# Autodesk Inventor assembly: Slidey Mecanum L thing
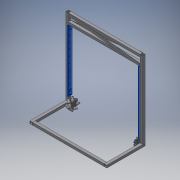
[picture p0: Inventor's stored thumbnail of the model, 180x180]
Saved by Autodesk Inventor 2018 (Build 220112000, 112)
## iProperties
Created: 2019-01-10
Part Number: Slidey Mecanum L thing
Document SubType Name: Assembly
Designer: maste
Author: maste
## Documents named in this file (8)
- C:\Users\maste\OneDrive\Documents\GitHub\2019CAD\Drivebase but Calvin is a mad man\Slidey Mecanum L thing.iam
- C:\Users\maste\OneDrive\Documents\GitHub\2019CAD\Drivebase but Calvin is a mad man\1x1 15in.ipt
- C:\Users\maste\OneDrive\Documents\GitHub\2019CAD\Drivebase but Calvin is a mad man\1x1 28 in.ipt
- C:\Users\maste\OneDrive\Documents\GitHub\2019CAD\Drivebase but Calvin is a mad man\1x1 30in.ipt
- C:\Users\maste\OneDrive\Documents\GitHub\2019CAD\Drivebase but Calvin is a mad man\4_Mecanum_Wheel_Left_217-3644.iam
- C:\Users\maste\OneDrive\Documents\GitHub\2019CAD\Drivebase but Calvin is a mad man\4_Mecanum_Wheel_Right_217-3645.iam
- C:\Users\maste\OneDrive\Documents\GitHub\2019CAD\Drivebase but Calvin is a mad man\User Library-plastic bearings_igus nk02-40-2-610.iam
- C:\Users\maste\OneDrive\Documents\GitHub\2019CAD\Drivebase but Calvin is a mad man\Strutural Integrity Bar.ipt
## Components (13 placed, 7 different names)
1. 1x1 15in:1 — Mate:1, Mate:2, Mate:3, Mate:10, Mate:11, Mate:12, Flush:1, Mate:18, Mate:19, Mate:20
2. 1x1 15in:2 — Mate:4, Mate:5, Mate:6, Mate:13, Mate:14, Mate:15, Mate:21, Mate:22, Mate:23
3. 1x1 28 in:1 — Mate:16, Mate:17, Flush:1, Mate:25, Mate:27
4. 1x1 28 in:2 — Mate:7, Mate:8, Mate:9, Mate:28, Mate:29, Mate:30, Mate:31
5. 1x1 28 in:3 — Mate:10, Mate:11, Mate:12, Mate:13, Mate:14, Mate:15
6. 1x1 30in:2 — Mate:1, Mate:2, Mate:3, Mate:7, Mate:8, Mate:9, Mate:16, Mate:17, Mate:24, Flush:2
7. 1x1 30in:3 — Mate:4, Mate:5, Mate:6, Mate:26, Flush:3
8. 4_Mecanum_Wheel_Left_217-3644:1 [sub-assembly] — Mate:21, Mate:22, Mate:23
9. 4_Mecanum_Wheel_Right_217-3645:1 [sub-assembly] — Mate:18, Mate:19, Mate:20
10. User Library-plastic bearings_igus nk02-40-2-610:1 [sub-assembly] — Mate:26, Mate:27, Flush:3
11. User Library-plastic bearings_igus nk02-40-2-610:2 [sub-assembly] — Mate:24, Mate:25, Flush:2
12. Strutural Integrity Bar:1 — Mate:28, Mate:29
13. Strutural Integrity Bar:2 — Mate:30, Mate:31
## Relationships (34: Mate 31, Flush 3)
- Mate:1: 1x1 15in:1 ↔ 1x1 30in:2
- Mate:2: 1x1 15in:1 ↔ 1x1 30in:2
- Mate:3: 1x1 15in:1 ↔ 1x1 30in:2
- Mate:4: 1x1 15in:2 ↔ 1x1 30in:3
- Mate:5: 1x1 15in:2 ↔ 1x1 30in:3
- Mate:6: 1x1 15in:2 ↔ 1x1 30in:3
- Mate:7: 1x1 28 in:2 ↔ 1x1 30in:2
- Mate:8: 1x1 28 in:2 ↔ 1x1 30in:2
- Mate:9: 1x1 28 in:2 ↔ 1x1 30in:2
- Mate:10: 1x1 15in:1 ↔ 1x1 28 in:3
- Mate:11: 1x1 15in:1 ↔ 1x1 28 in:3
- Mate:12: 1x1 15in:1 ↔ 1x1 28 in:3
- Mate:13: 1x1 15in:2 ↔ 1x1 28 in:3
- Mate:14: 1x1 15in:2 ↔ 1x1 28 in:3
- Mate:15: 1x1 15in:2 ↔ 1x1 28 in:3
- Mate:16: 1x1 28 in:1 ↔ 1x1 30in:2
- Mate:17: 1x1 28 in:1 ↔ 1x1 30in:2
- Flush:1 (685.8 mm): 1x1 15in:1 ↔ 1x1 28 in:1
- Mate:18: 1x1 15in:1 ↔ 4_Mecanum_Wheel_Right_217-3645:1
- Mate:19: 1x1 15in:1 ↔ 4_Mecanum_Wheel_Right_217-3645:1
- Mate:20: 1x1 15in:1 ↔ 4_Mecanum_Wheel_Right_217-3645:1
- Mate:21: 1x1 15in:2 ↔ 4_Mecanum_Wheel_Left_217-3644:1
- Mate:22: 1x1 15in:2 ↔ 4_Mecanum_Wheel_Left_217-3644:1
- Mate:23: 1x1 15in:2 ↔ 4_Mecanum_Wheel_Left_217-3644:1
- Mate:24: 1x1 30in:2 ↔ User Library-plastic bearings_igus nk02-40-2-610:2
- Mate:25: 1x1 28 in:1 ↔ User Library-plastic bearings_igus nk02-40-2-610:2
- Flush:2 (-10.0012 mm): 1x1 30in:2 ↔ User Library-plastic bearings_igus nk02-40-2-610:2
- Mate:26: 1x1 30in:3 ↔ User Library-plastic bearings_igus nk02-40-2-610:1
- Mate:27: 1x1 28 in:1 ↔ User Library-plastic bearings_igus nk02-40-2-610:1
- Flush:3 (-10.0012 mm): 1x1 30in:3 ↔ User Library-plastic bearings_igus nk02-40-2-610:1
- Mate:28: 1x1 28 in:2 ↔ Strutural Integrity Bar:1
- Mate:29: 1x1 28 in:2 ↔ Strutural Integrity Bar:1
- Mate:30: 1x1 28 in:2 ↔ Strutural Integrity Bar:2
- Mate:31: 1x1 28 in:2 ↔ Strutural Integrity Bar:2
